# Autodesk Inventor assembly: Elevator MK2
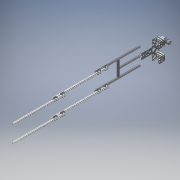
[picture p0: Inventor's stored thumbnail of the model, 180x180]
Saved by Autodesk Inventor 2019.4 (Build 234330000, 330)
## iProperties
Created: 2020-01-23
Part Number: Elevator MK2
Document SubType Name: Assembly
Designer: Mark
Mass: 1724.74 g
Surface Area: 8260.68 cm^2
Volume: 882.165 cm^3
Density: 1.95512 g/cm^3
Author: Mark
## Documents named in this file (8)
- C:\Users\Mark\Desktop\7738 Helion Engineering\7738-2020\Elevator MK2\Elevator MK2.iam
- C:\Users\Mark\Desktop\7738 Helion Engineering\7738-2020\Spinny disk assembly\Aluminium extrusion profile 2020.ipt
- C:\Users\Mark\Desktop\7738 Helion Engineering\7738-2020\Elevator MK2\Mini V Gantry Kit.ipt
- C:\Users\Mark\Desktop\7738 Helion Engineering\7738-2020\Elevator MK2\Second Stage  Extrusion.ipt
- C:\Users\Mark\Desktop\7738 Helion Engineering\7738-2020\Elevator MK2\Final Stage.ipt
- C:\Users\Mark\Desktop\7738 Helion Engineering\7738-2020\Elevator MK2\Final Extrusion Mid.ipt
- **C:\Users\Mark\Desktop\7738 Helion Engineering\7738-2020\Robot Assembly MK2.iam*LocalDocs*x2tom4pch4vblelovMqgcvgtxXa*AdjusterAssembly.iam
- C:\Users\Mark\Desktop\7738 Helion Engineering\7738-2020\Elevator MK2\Up extrusion.ipt
## Components (17 placed, 7 different names)
1. Aluminium extrusion profile 2020:1 — Flush:1, Flush:2, Mate:1, Flush:17
2. Aluminium extrusion profile 2020:2 — Flush:1, Flush:2, Mate:1, Flush:20, Mate:23
3. Mini V Gantry Kit:1 — Mate:12, Mate:13, Mate:14
4. Mini V Gantry Kit:2 — Mate:27, Mate:28, Mate:29
5. Mini V Gantry Kit:3 — Mate:24, Mate:25, Mate:26
6. Mini V Gantry Kit:4 — Mate:15, Mate:16, Mate:17
7. Second Stage  Extrusion:1 — Mate:12, Mate:13, Mate:14, Mate:15, Mate:16, Mate:17, Flush:17, Mate:19, Flush:18, Flush:19
8. Second Stage  Extrusion:2 — Mate:19, Flush:18, Flush:19, Mate:20, Mate:21, Mate:22, Flush:20, Mate:23, Flush:23, Mate:37
9. Final Stage:1 — Mate:24, Mate:25, Mate:26, Mate:27, Mate:28, Mate:29, Flush:21, Flush:22, Flush:23, Mate:37, Mate:38, Flush:24, Mate:39, Flush:25, Mate:41
10. Mini V Gantry Kit:5 — Mate:20, Mate:21, Mate:22
11. Mini V Gantry Kit:8
12. Mini V Gantry Kit:9
13. Mini V Gantry Kit:10
14. Final Stage:2 — Flush:21, Flush:22, Mate:38
15. Final Extrusion Mid:1 — Flush:24, Mate:39, Flush:25, Mate:40, Flush:26
16. AdjusterAssembly:1 [sub-assembly] — Mate:42, Flush:27
17. Up extrusion:1 — Mate:40, Flush:26, Mate:41, Mate:42, Flush:27
## Relationships (46: Mate 31, Flush 15)
- Flush:1: Aluminium extrusion profile 2020:1 ↔ Aluminium extrusion profile 2020:2
- Flush:2: Aluminium extrusion profile 2020:1 ↔ Aluminium extrusion profile 2020:2
- Mate:1 (200 mm): Aluminium extrusion profile 2020:1 ↔ Aluminium extrusion profile 2020:2
- [Flush]: Mini V Gantry Kit:5 ↔ Mini V Gantry Kit:8
- [Flush]: Mini V Gantry Kit:5 ↔ Mini V Gantry Kit:8
- [Mate] (50 mm): Mini V Gantry Kit:5 ↔ Mini V Gantry Kit:8
- Mate:12: Mini V Gantry Kit:1 ↔ Second Stage  Extrusion:1
- Mate:13: Mini V Gantry Kit:1 ↔ Second Stage  Extrusion:1
- Mate:14: Mini V Gantry Kit:1 ↔ Second Stage  Extrusion:1
- Mate:15: Mini V Gantry Kit:4 ↔ Second Stage  Extrusion:1
- Mate:16: Mini V Gantry Kit:4 ↔ Second Stage  Extrusion:1
- Mate:17: Mini V Gantry Kit:4 ↔ Second Stage  Extrusion:1
- Flush:17: Aluminium extrusion profile 2020:1 ↔ Second Stage  Extrusion:1
- Mate:19 (200 mm): Second Stage  Extrusion:1 ↔ Second Stage  Extrusion:2
- Flush:18: Second Stage  Extrusion:1 ↔ Second Stage  Extrusion:2
- Flush:19: Second Stage  Extrusion:1 ↔ Second Stage  Extrusion:2
- Mate:20: Second Stage  Extrusion:2 ↔ Mini V Gantry Kit:5
- Mate:21: Second Stage  Extrusion:2 ↔ Mini V Gantry Kit:5
- Mate:22: Second Stage  Extrusion:2 ↔ Mini V Gantry Kit:5
- Flush:20: Aluminium extrusion profile 2020:2 ↔ Second Stage  Extrusion:2
- Mate:23 (6.4 mm): Aluminium extrusion profile 2020:2 ↔ Second Stage  Extrusion:2
- Mate:24: Mini V Gantry Kit:3 ↔ Final Stage:1
- Mate:25: Mini V Gantry Kit:3 ↔ Final Stage:1
- Mate:26: Mini V Gantry Kit:3 ↔ Final Stage:1
- Mate:27: Mini V Gantry Kit:2 ↔ Final Stage:1
- Mate:28: Mini V Gantry Kit:2 ↔ Final Stage:1
- Mate:29: Mini V Gantry Kit:2 ↔ Final Stage:1
- [Mate]: Mini V Gantry Kit:10 ↔ Final Stage:2
- [Mate]: Mini V Gantry Kit:10 ↔ Final Stage:2
- [Mate]: Mini V Gantry Kit:10 ↔ Final Stage:2
- [Mate]: Mini V Gantry Kit:9 ↔ Final Stage:2
- [Mate]: Mini V Gantry Kit:9 ↔ Final Stage:2
- [Mate]: Mini V Gantry Kit:9 ↔ Final Stage:2
- Flush:21: Final Stage:1 ↔ Final Stage:2
- Flush:22: Final Stage:1 ↔ Final Stage:2
- Flush:23: Second Stage  Extrusion:2 ↔ Final Stage:1
- Mate:37 (6.4 mm): Second Stage  Extrusion:2 ↔ Final Stage:1
- Mate:38 (200 mm): Final Stage:1 ↔ Final Stage:2
- Flush:24 (280 mm): Final Stage:1 ↔ Final Extrusion Mid:1
- Mate:39: Final Stage:1 ↔ Final Extrusion Mid:1
- Flush:25: Final Stage:1 ↔ Final Extrusion Mid:1
- Mate:40: Final Extrusion Mid:1 ↔ Up extrusion:1
- Flush:26: Final Extrusion Mid:1 ↔ Up extrusion:1
- Mate:41 (90 mm): Final Stage:1 ↔ Up extrusion:1
- Mate:42 (0.4 mm): AdjusterAssembly:1 ↔ Up extrusion:1
- Flush:27 (-15 mm): AdjusterAssembly:1 ↔ Up extrusion:1
## Named parameters: d22_d13 = 50 mm, d25_d48 = 0 mm, d26_d49 = 0 mm, d51_d45 = 0 mm, d52_d46 = 0 mm, d53_d47 = 0 mm, d54_d48 = 0 mm, d55_d49 = 0 mm, d56_d50 = 0 mm
